# Autodesk Inventor assembly: Benchmark
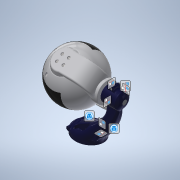
[picture p0: Inventor's stored thumbnail of the model, 180x180]
Saved by Autodesk Inventor 2021.1 (Build 251245010, 245A)
## iProperties
Part Number: Benchmark
Material: Типовые
Document SubType Name: Assembly
Designer: stud
Author: stud
## Documents named in this file (21)
- C:\bkp\FYPDESIGN\Benchmark.iam
- C:\Users\Drake\Downloads\cctv-camera-5.snapshot.3\Kamera.ipt
- C:\Users\Drake\Downloads\cctv-camera-5.snapshot.3\Dvigatel.ipt
- C:\Users\Drake\Downloads\cctv-camera-5.snapshot.3\Держатель.ipt
- C:\Users\Drake\Downloads\cctv-camera-5.snapshot.3\Корпус камеры.ipt
- C:\Users\Drake\Downloads\cctv-camera-5.snapshot.3\ДержательКорпКам.ipt
- C:\Users\Drake\Downloads\cctv-camera-5.snapshot.3\Держатель_КОПИЯ.ipt
- C:\Users\Drake\Downloads\cctv-camera-5.snapshot.3\Держатель_КОПИЯ_ЗЕРКАЛО.ipt
- C:\Users\Drake\Downloads\cctv-camera-5.snapshot.3\ДержательКорпКамЧ.1.ipt
- C:\Users\Drake\Downloads\cctv-camera-5.snapshot.3\ДержательКорпКамЧ.2.ipt
- C:\Users\Drake\Downloads\cctv-camera-5.snapshot.3\Винт M2.5-6gx8 ГОСТ Р 50405-92.ipt
- C:\Users\Drake\Downloads\cctv-camera-5.snapshot.3\Винт M3-6gx25 ГОСТ Р 50405-92.ipt
- C:\Users\Drake\Downloads\cctv-camera-5.snapshot.3\Винт M3-6gx22 ГОСТ Р 50405-92.ipt
- C:\Users\Drake\Downloads\cctv-camera-5.snapshot.3\Винт M3-6gx11 ГОСТ Р 50405-92.ipt
- C:\Users\Drake\Downloads\cctv-camera-5.snapshot.3\Кронштейн.ipt
- C:\Users\Drake\Downloads\cctv-camera-5.snapshot.3\Кронштейн_ЗЕРКАЛО.ipt
- C:\Users\Drake\Downloads\cctv-camera-5.snapshot.3\Корпус камерыЧ2.ipt
- C:\Users\Drake\Downloads\cctv-camera-5.snapshot.3\Винт A M2-6gx8 ГОСТ Р 50404-92.ipt
- C:\Users\Drake\Downloads\cctv-camera-5.snapshot.3\Винт A2.M1.6-6gx13 ГОСТ Р 50403-92.ipt
- C:\Users\Drake\Downloads\cctv-camera-5.snapshot.3\Винт A2.M1.6-6gx6 ГОСТ Р 50403-92.ipt
- C:\Users\Drake\Downloads\cctv-camera-5.snapshot.3\Винт A2.M2-6gx11 ГОСТ Р 50403-92.ipt
## Components (30 placed, 20 different names)
1. Kamera:1 — Совмещение:16, Совмещение:17, Совмещение:18, Совмещение:19, Заподлицо:5, Заподлицо:6, Совмещение:20, Совмещение:21, Заподлицо:7, Заподлицо:10
2. Dvigatel:1 — Совмещение:5, Заподлицо:4, Угол:1, Совмещение:13
3. Держатель:1 — Совмещение:1, Заподлицо:2, Заподлицо:3, Совмещение:5, Заподлицо:4
4. Корпус камеры:1 — Совмещение:20, Совмещение:21, Заподлицо:7, Совмещение:22 Сдвиг Y, Заподлицо:8, Совмещение:23, Совмещение:24, Совмещение:25, Совмещение:26, Совмещение:27, Совмещение:33, Совмещение:34, Заподлицо:9, Совмещение:37, Совмещение:38
5. ДержательКорпКам:1
6. Держатель_КОПИЯ:1
7. Держатель_КОПИЯ_ЗЕРКАЛО:1 — Совмещение:1, Заподлицо:2, Заподлицо:3, Вставка:1, Вставка:2, Совмещение:3, Совмещение:4, Совмещение:14
8. Винт M3-6gx25 ГОСТ Р 50405-92:1 — Вставка:1
9. Винт M3-6gx22 ГОСТ Р 50405-92:1 — Вставка:2
10. Винт M3-6gx11 ГОСТ Р 50405-92:1 — Совмещение:3, Совмещение:4
11. ДержательКорпКамЧ.1:1 — Совмещение:6, Совмещение:7, Совмещение:8, Совмещение:13, Совмещение:14, Совмещение:15, Допуск симметричности:1, Угол:4, Заподлицо:8, Совмещение:24, Совмещение:25, Вставка:3, Вставка:4, Вставка:5, Вставка:6
12. ДержательКорпКамЧ.2:1 — Совмещение:6, Совмещение:7, Совмещение:8, Совмещение:9, Совмещение:10, Совмещение:11, Совмещение:12, Допуск симметричности:1, Совмещение:23, Совмещение:26, Совмещение:27
13. Винт M2.5-6gx8 ГОСТ Р 50405-92:1 — Совмещение:9, Совмещение:11
14. Винт M2.5-6gx8 ГОСТ Р 50405-92:2 — Совмещение:10, Совмещение:12
15. Кронштейн:1 — Совмещение:18, Совмещение:19, Заподлицо:5, Совмещение:29, Совмещение:30
16. Кронштейн_ЗЕРКАЛО:1 — Совмещение:16, Совмещение:17, Заподлицо:6, Совмещение:31, Совмещение:32
17. Корпус камерыЧ2:1 — Совмещение:33, Совмещение:34, Заподлицо:9, Заподлицо:10, Совмещение:35, Совмещение:36
18. Винт A M2-6gx8 ГОСТ Р 50404-92:1 — Вставка:3
19. Винт A M2-6gx8 ГОСТ Р 50404-92:2 — Вставка:4
20. Винт A M2-6gx8 ГОСТ Р 50404-92:3 — Вставка:5
21. Винт A M2-6gx8 ГОСТ Р 50404-92:4 — Вставка:6
22. Винт A2.M1.6-6gx13 ГОСТ Р 50403-92:1
23. Винт A2.M1.6-6gx6 ГОСТ Р 50403-92:1 — Совмещение:29
24. Винт A2.M1.6-6gx6 ГОСТ Р 50403-92:2 — Совмещение:30
25. Винт A2.M1.6-6gx6 ГОСТ Р 50403-92:3 — Совмещение:31
26. Винт A2.M1.6-6gx6 ГОСТ Р 50403-92:4 — Совмещение:32
27. Винт A2.M2-6gx11 ГОСТ Р 50403-92:1 — Совмещение:35
28. Винт A2.M2-6gx11 ГОСТ Р 50403-92:2 — Совмещение:36
29. Винт A2.M2-6gx11 ГОСТ Р 50403-92:3 — Совмещение:37
30. Винт A2.M2-6gx11 ГОСТ Р 50403-92:4 — Совмещение:38
## Relationships (56: Mate 37, Flush 9, Insert 6, Angle 3, Symmetry 1)
- Совмещение:1 [Mate]: Держатель:1 ↔ Держатель_КОПИЯ_ЗЕРКАЛО:1
- Заподлицо:2 [Flush]: Держатель:1 ↔ Держатель_КОПИЯ_ЗЕРКАЛО:1
- Заподлицо:3 [Flush]: Держатель:1 ↔ Держатель_КОПИЯ_ЗЕРКАЛО:1
- Вставка:1 [Insert]: Держатель_КОПИЯ_ЗЕРКАЛО:1 ↔ Винт M3-6gx25 ГОСТ Р 50405-92:1
- Вставка:2 [Insert]: Держатель_КОПИЯ_ЗЕРКАЛО:1 ↔ Винт M3-6gx22 ГОСТ Р 50405-92:1
- Совмещение:3 [Mate]: Держатель_КОПИЯ_ЗЕРКАЛО:1 ↔ Винт M3-6gx11 ГОСТ Р 50405-92:1
- Совмещение:4 [Mate]: Держатель_КОПИЯ_ЗЕРКАЛО:1 ↔ Винт M3-6gx11 ГОСТ Р 50405-92:1
- Совмещение:5 [Mate]: Dvigatel:1 ↔ Держатель:1
- Заподлицо:4 [Flush]: Dvigatel:1 ↔ Держатель:1
- Угол:1 [Angle] (180 deg): Dvigatel:1
- Совмещение:6 [Mate]: ДержательКорпКамЧ.1:1 ↔ ДержательКорпКамЧ.2:1
- Совмещение:7 [Mate]: ДержательКорпКамЧ.1:1 ↔ ДержательКорпКамЧ.2:1
- Совмещение:8 [Mate]: ДержательКорпКамЧ.1:1 ↔ ДержательКорпКамЧ.2:1
- Совмещение:9 [Mate]: ДержательКорпКамЧ.2:1 ↔ Винт M2.5-6gx8 ГОСТ Р 50405-92:1
- Совмещение:10 [Mate]: ДержательКорпКамЧ.2:1 ↔ Винт M2.5-6gx8 ГОСТ Р 50405-92:2
- Совмещение:11 [Mate]: ДержательКорпКамЧ.2:1 ↔ Винт M2.5-6gx8 ГОСТ Р 50405-92:1
- Совмещение:12 [Mate]: ДержательКорпКамЧ.2:1 ↔ Винт M2.5-6gx8 ГОСТ Р 50405-92:2
- Совмещение:13 [Mate]: Dvigatel:1 ↔ ДержательКорпКамЧ.1:1
- Совмещение:14 [Mate] (0.5 mm): Держатель_КОПИЯ_ЗЕРКАЛО:1 ↔ ДержательКорпКамЧ.1:1
- Совмещение:15 [Mate]: ДержательКорпКамЧ.1:1
- Угол:2 [Angle] (0 deg)
- Допуск симметричности:1 [Symmetry]: ДержательКорпКамЧ.1:1 ↔ ДержательКорпКамЧ.2:1
- Угол:4 [Angle] (0 deg): ДержательКорпКамЧ.1:1
- Совмещение:16 [Mate]: Kamera:1 ↔ Кронштейн_ЗЕРКАЛО:1
- Совмещение:17 [Mate]: Kamera:1 ↔ Кронштейн_ЗЕРКАЛО:1
- Совмещение:18 [Mate]: Kamera:1 ↔ Кронштейн:1
- Совмещение:19 [Mate]: Kamera:1 ↔ Кронштейн:1
- Заподлицо:5 [Flush]: Kamera:1 ↔ Кронштейн:1
- Заподлицо:6 [Flush]: Kamera:1 ↔ Кронштейн_ЗЕРКАЛО:1
- Совмещение:20 [Mate]: Kamera:1 ↔ Корпус камеры:1
- Совмещение:21 [Mate]: Kamera:1 ↔ Корпус камеры:1
- Заподлицо:7 [Flush]: Kamera:1 ↔ Корпус камеры:1
- Совмещение:22 Сдвиг Y [Mate] (1.5 mm): Корпус камеры:1
- Заподлицо:8 [Flush]: Корпус камеры:1 ↔ ДержательКорпКамЧ.1:1
- Совмещение:23 [Mate]: Корпус камеры:1 ↔ ДержательКорпКамЧ.2:1
- Совмещение:24 [Mate]: Корпус камеры:1 ↔ ДержательКорпКамЧ.1:1
- Совмещение:25 [Mate]: Корпус камеры:1 ↔ ДержательКорпКамЧ.1:1
- Совмещение:26 [Mate]: Корпус камеры:1 ↔ ДержательКорпКамЧ.2:1
- Совмещение:27 [Mate]: Корпус камеры:1 ↔ ДержательКорпКамЧ.2:1
- Вставка:3 [Insert]: ДержательКорпКамЧ.1:1 ↔ Винт A M2-6gx8 ГОСТ Р 50404-92:1
- Вставка:4 [Insert]: ДержательКорпКамЧ.1:1 ↔ Винт A M2-6gx8 ГОСТ Р 50404-92:2
- Вставка:5 [Insert]: ДержательКорпКамЧ.1:1 ↔ Винт A M2-6gx8 ГОСТ Р 50404-92:3
- Вставка:6 [Insert]: ДержательКорпКамЧ.1:1 ↔ Винт A M2-6gx8 ГОСТ Р 50404-92:4
- [Mate]: ДержательКорпКамЧ.2:1 ↔ Винт A2.M1.6-6gx13 ГОСТ Р 50403-92:1
- Совмещение:29 [Mate]: Кронштейн:1 ↔ Винт A2.M1.6-6gx6 ГОСТ Р 50403-92:1
- Совмещение:30 [Mate]: Кронштейн:1 ↔ Винт A2.M1.6-6gx6 ГОСТ Р 50403-92:2
- Совмещение:31 [Mate]: Кронштейн_ЗЕРКАЛО:1 ↔ Винт A2.M1.6-6gx6 ГОСТ Р 50403-92:3
- Совмещение:32 [Mate]: Кронштейн_ЗЕРКАЛО:1 ↔ Винт A2.M1.6-6gx6 ГОСТ Р 50403-92:4
- Совмещение:33 [Mate]: Корпус камеры:1 ↔ Корпус камерыЧ2:1
- Совмещение:34 [Mate]: Корпус камеры:1 ↔ Корпус камерыЧ2:1
- Заподлицо:9 [Flush]: Корпус камеры:1 ↔ Корпус камерыЧ2:1
- Заподлицо:10 [Flush]: Kamera:1 ↔ Корпус камерыЧ2:1
- Совмещение:35 [Mate]: Корпус камерыЧ2:1 ↔ Винт A2.M2-6gx11 ГОСТ Р 50403-92:1
- Совмещение:36 [Mate]: Корпус камерыЧ2:1 ↔ Винт A2.M2-6gx11 ГОСТ Р 50403-92:2
- Совмещение:37 [Mate]: Корпус камеры:1 ↔ Винт A2.M2-6gx11 ГОСТ Р 50403-92:3
- Совмещение:38 [Mate]: Корпус камеры:1 ↔ Винт A2.M2-6gx11 ГОСТ Р 50403-92:4
